# Autodesk Inventor assembly: Extruder Carriage
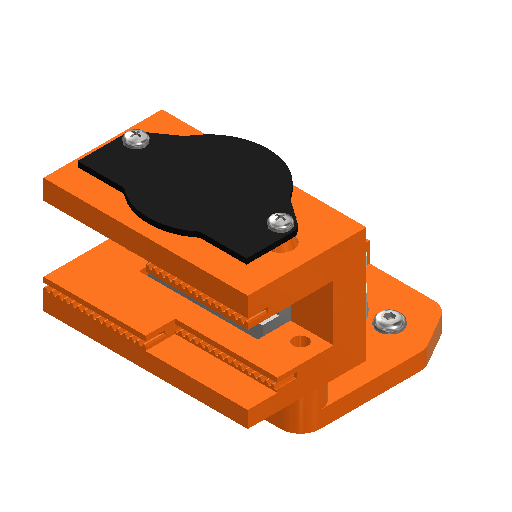
[picture p0: Inventor's stored thumbnail of the model, 512x512]
Saved by Autodesk Inventor 2023.2 (Build 272271000, 271)
## iProperties
Created: 2023-02-03
Part Number: Extruder Carriage
Document SubType Name: Assembly
Designer: remop
Author: remop
## Documents named in this file (8)
- C:\Users\remop\OneDrive\Documents\Inventor\3D Printers\LuEVO\Mk5_FullKinematic\Extruder Carriage.iam
- C:\Users\remop\OneDrive\Documents\Inventor\3D Printers\LuEVO\Mk5_FullKinematic\MGN12C.ipt
- C:\Users\remop\OneDrive\Documents\Inventor\3D Printers\LuEVO\Mk4_Toolchanger\final_Toolhead.iam
- C:\Users\remop\OneDrive\Documents\Inventor\3D Printers\LuEVO\Mk5_FullKinematic\Toolhead Base.ipt
- C:\Users\remop\OneDrive\Documents\Inventor\Content Center Files\R2023\en-US\AS 1427(04)\AS 1427 - M5 x 16(5) I.ipt
- C:\Users\remop\OneDrive\Documents\Inventor\Content Center Files\R2023\en-US\AS 1420\AS 1420 - 1973 - M3 x 8.ipt
- C:\Users\remop\OneDrive\Documents\Inventor\3D Printers\LuEVO\Mk5_FullKinematic\Mellow Fly SHT36.ipt
- C:\Users\remop\OneDrive\Documents\Inventor\Content Center Files\R2023\en-US\AS 1427(05)\AS 1427 - M3 x 5(5) II.ipt
## Components (11 placed, 7 different names)
1. MGN12C:1 — Mate:1, Mate:2, Flush:1
2. final_Toolhead:1 [sub-assembly] — Mate:1, Mate:2, Flush:1, Flush:2, Rotational:1, Rotational:2
3. Toolhead Base:1 — Flush:2, Insert:1, Insert:2, Insert:3, Flush:3, Mate:3, Flush:4
4. AS 1427 H - Metric M5 x 16:1 — Rotational:2
5. AS 1427 H - Metric M5 x 16:2 — Rotational:1
6. AS 1420 - Metric M3 x 8:1 — Insert:1
7. AS 1420 - Metric M3 x 8:2 — Insert:2
8. AS 1420 - Metric M3 x 8:3 — Insert:3
9. Mellow Fly SHT36:1 — Flush:3, Mate:3, Flush:4, Insert:4, Insert:5
10. AS 1427 H - Metric M3 x 5:1 — Insert:4
11. AS 1427 H - Metric M3 x 5:2 — Insert:5
## Relationships (14: Insert 5, Flush 4, Mate 3, RevoluteJoint 2)
- Mate:1 (4 mm): MGN12C:1 ↔ final_Toolhead:1
- Mate:2 (-12 mm): MGN12C:1 ↔ final_Toolhead:1
- Flush:1 (13.795 mm): MGN12C:1 ↔ final_Toolhead:1
- Flush:2: final_Toolhead:1 ↔ Toolhead Base:1
- Rotational:1 [RevoluteJoint]: final_Toolhead:1 ↔ AS 1427 H - Metric M5 x 16:2
- Rotational:2 [RevoluteJoint]: final_Toolhead:1 ↔ AS 1427 H - Metric M5 x 16:1
- Insert:1: Toolhead Base:1 ↔ AS 1420 - Metric M3 x 8:1
- Insert:2: Toolhead Base:1 ↔ AS 1420 - Metric M3 x 8:2
- Insert:3: Toolhead Base:1 ↔ AS 1420 - Metric M3 x 8:3
- Flush:3 (5 mm): Toolhead Base:1 ↔ Mellow Fly SHT36:1
- Mate:3 (3 mm): Toolhead Base:1 ↔ Mellow Fly SHT36:1
- Flush:4 (5.365 mm): Toolhead Base:1 ↔ Mellow Fly SHT36:1
- Insert:4: Mellow Fly SHT36:1 ↔ AS 1427 H - Metric M3 x 5:1
- Insert:5: Mellow Fly SHT36:1 ↔ AS 1427 H - Metric M3 x 5:2
